# Autodesk Inventor assembly: Leg_joint_roll_pitch
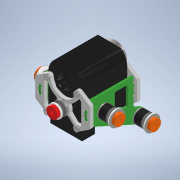
[picture p0: Inventor's stored thumbnail of the model, 180x180]
Saved by Autodesk Inventor 2020 (Build 240168000, 168)
## iProperties
Part Number: Leg_joint_roll_pitch
Document SubType Name: Assembly
Designer: Masato Kubotera
Mass: 101.309 g
Surface Area: 368.925 cm^2
Volume: 74.117 cm^3
Density: 1.36688 g/cm^3
Author: Masato Kubotera
## Documents named in this file (20)
- C:\Users\MasatoKubotera\Documents\Inventor\SUSTAINA-OP\LowerBody\Leg_joint\Leg_joint_roll_pitch.iam
- C:\Users\MasatoKubotera\Documents\Inventor\SUSTAINA-OP\LowerBody\Leg_joint\Leg_joint_pitch_frame.ipt
- C:\Users\MasatoKubotera\Documents\Inventor\SUSTAINA-OP\LowerBody\Leg_joint\Leg_joint_roll_frame.ipt
- C:\Users\MasatoKubotera\Documents\Inventor\SUSTAINA-OP\ReadyMade\Screw\M2_6-20.ipt
- C:\Users\MasatoKubotera\Documents\Inventor\SUSTAINA-OP\ReadyMade\Screw\M2_6-15.ipt
- C:\Users\MasatoKubotera\Documents\Inventor\SUSTAINA-OP\ReadyMade\Bush\80F-0603.ipt
- C:\Users\MasatoKubotera\Documents\Inventor\SUSTAINA-OP\ReadyMade\Washer\CC-0612-50B.ipt
- C:\Users\MasatoKubotera\Documents\Inventor\SUSTAINA-OP\ReadyMade\InsertNut\SF419.ipt
- C:\Users\MasatoKubotera\Documents\Inventor\SUSTAINA-OP\ReadyMade\Washer\UUW-0412-10H.ipt
- C:\Users\MasatoKubotera\Documents\Inventor\SUSTAINA-OP\ReadyMade\Spacer\SLSBF6-39.5-M4-N4.ipt
- C:\Users\MasatoKubotera\Documents\Inventor\SUSTAINA-OP\ReadyMade\Screw\DBTS4-11-6-DHC.ipt
- C:\Users\MasatoKubotera\Documents\Inventor\SUSTAINA-OP\ReadyMade\Screw\DBTS4-5-5-DHC.ipt
- C:\Users\MasatoKubotera\Documents\Inventor\SUSTAINA-OP\ReadyMade\Screw\DBTS4-10-4-DHC.ipt
- C:\Users\MasatoKubotera\Documents\Inventor\SUSTAINA-OP\ReadyMade\InsertNut\S4-05-3W.ipt
- C:\Users\MasatoKubotera\Documents\Inventor\SUSTAINA-OP\ReadyMade\Screw\DBTS4-11-8-DHC.ipt
- C:\Users\MasatoKubotera\Documents\Inventor\SUSTAINA-OP\ReadyMade\Washer\TT-0612-10.ipt
- C:\Users\MasatoKubotera\Documents\Inventor\SUSTAINA-OP\ReadyMade\Washer\TT-0814-10.ipt
- C:\Users\MasatoKubotera\Documents\Inventor\SUSTAINA-OP\ReadyMade\Washer\CCC-0612-65B.ipt
- C:\Users\MasatoKubotera\Documents\Inventor\SUSTAINA-OP\ReadyMade\KONDO\B3M-SC-1170-A_with_ClampHorn.iam
- C:\Users\MasatoKubotera\Documents\Inventor\SUSTAINA-OP\ReadyMade\Washer\UUW-0614-03H.ipt
## Components (50 placed, 19 different names)
1. B3M-SC-1170-A_with_ClampHorn:1 [sub-assembly] — 挿入:246, 挿入:247, 挿入:248, 挿入:249, メイト:18, フラッシュ:10, メイト:19
2. Leg_joint_roll_frame:1 — 挿入:5, 挿入:6, 挿入:7, 挿入:8, 挿入:9, 挿入:10, 角度:1, フラッシュ:2, メイト:3, メイト:4, メイト:5, 挿入:248, 挿入:249
3. Leg_joint_roll_frame:2 — 挿入:15, 挿入:16, 挿入:17, 挿入:18, 角度:2, 角度:4, 挿入:246, 挿入:247
4. Leg_joint_pitch_frame:1 — フラッシュ:3, 挿入:19, フラッシュ:4, メイト:5, 挿入:20, 挿入:21, 挿入:22
5. Leg_joint_pitch_frame:2 — フラッシュ:2, フラッシュ:3, フラッシュ:4, メイト:3, メイト:4, 挿入:23, 挿入:24, 挿入:25, 挿入:26
6. UUW-0412-10H:1 — 挿入:9, 挿入:27
7. UUW-0412-10H:2 — 挿入:17, 挿入:28, 挿入:33
8. UUW-0412-10H:3 — 挿入:19, 挿入:226, 挿入:241
9. UUW-0412-10H:4 — 挿入:22, 挿入:35, 挿入:240
10. UUW-0412-10H:5 — 挿入:23, 挿入:227, 挿入:239
11. UUW-0412-10H:6 — 挿入:26, 挿入:37, 挿入:238
12. UUW-0412-10H:7 — 挿入:27, 挿入:38, 挿入:43
13. SF419:1 — 挿入:25
14. SF419:2 — 挿入:20
15. S4-05-3W:1 — 挿入:10, 角度:1
16. S4-05-3W:2 — 挿入:18, 角度:2
17. SLSBF6-39.5-M4-N4:1 — 挿入:21, 挿入:24, 角度:4
18. DBS4-5-5:1 — 挿入:38, 挿入:232
19. DBTS4-11-6:3 — 挿入:37, 挿入:257
20. DBTS4-11-6:4 — 挿入:35, 挿入:254
21. DBTS4-10-4:1 — 挿入:33, 挿入:233
22. DBTS4-11-8:1 — 挿入:226, 挿入:255
23. DBTS4-11-8:2 — 挿入:227, 挿入:256
24. TT-0612-10:1 — 挿入:233
25. TT-0612-10:2 — 挿入:232
26. TT-0814-10:1 — 挿入:250
27. TT-0814-10:2 — 挿入:251
28. TT-0814-10:3 — 挿入:253
29. TT-0814-10:4 — 挿入:252
30. CCC-0612-65B:1 — 挿入:238, 挿入:245
31. CCC-0612-65B:2 — 挿入:241, 挿入:243
32. CCC-0612-65B:3 — 挿入:239, 挿入:244
33. CCC-0612-65B:4 — 挿入:240, 挿入:242
34. CC-0612-50B:5 — 挿入:28, 挿入:44
35. 80F-0603:1 — 挿入:43
36. 80F-0603:2 — 挿入:44
37. 80F-0603:3 — 挿入:243
38. 80F-0603:4 — 挿入:242
39. 80F-0603:5 — 挿入:244
40. 80F-0603:6 — 挿入:245
41. UUW-0614-03H:1 — 挿入:250, 挿入:256
42. UUW-0614-03H:2 — 挿入:251, 挿入:257
43. UUW-0614-03H:3 — 挿入:253, 挿入:255
44. UUW-0614-03H:4 — 挿入:252, 挿入:254
45. M2_6-20:1 — 挿入:7
46. M2_6-20:2 — 挿入:8
47. M2_6-20:3 — 挿入:5
48. M2_6-20:4 — 挿入:6
49. M2_6-15:2 — 挿入:16
50. M2_6-15:3 — 挿入:15
## Relationships (62: Insert 50, Mate 5, Flush 4, Angle 3)
- 挿入:5 [Insert]: Leg_joint_roll_frame:1 ↔ M2_6-20:3
- 挿入:6 [Insert]: Leg_joint_roll_frame:1 ↔ M2_6-20:4
- 挿入:7 [Insert]: Leg_joint_roll_frame:1 ↔ M2_6-20:1
- 挿入:8 [Insert]: Leg_joint_roll_frame:1 ↔ M2_6-20:2
- 挿入:9 [Insert]: Leg_joint_roll_frame:1 ↔ UUW-0412-10H:1
- 挿入:10 [Insert]: Leg_joint_roll_frame:1 ↔ S4-05-3W:1
- 角度:1 [Angle] (0 deg): Leg_joint_roll_frame:1 ↔ S4-05-3W:1
- 挿入:15 [Insert]: Leg_joint_roll_frame:2 ↔ M2_6-15:3
- 挿入:16 [Insert]: Leg_joint_roll_frame:2 ↔ M2_6-15:2
- 挿入:17 [Insert]: Leg_joint_roll_frame:2 ↔ UUW-0412-10H:2
- 挿入:18 [Insert]: Leg_joint_roll_frame:2 ↔ S4-05-3W:2
- 角度:2 [Angle] (0 deg): Leg_joint_roll_frame:2 ↔ S4-05-3W:2
- 挿入:19 [Insert]: Leg_joint_pitch_frame:1 ↔ UUW-0412-10H:3
- 挿入:20 [Insert]: Leg_joint_pitch_frame:1 ↔ SF419:2
- 挿入:21 [Insert]: Leg_joint_pitch_frame:1 ↔ SLSBF6-39.5-M4-N4:1
- 挿入:22 [Insert]: Leg_joint_pitch_frame:1 ↔ UUW-0412-10H:4
- 挿入:23 [Insert]: Leg_joint_pitch_frame:2 ↔ UUW-0412-10H:5
- 挿入:24 [Insert]: Leg_joint_pitch_frame:2 ↔ SLSBF6-39.5-M4-N4:1
- 挿入:25 [Insert]: Leg_joint_pitch_frame:2 ↔ SF419:1
- 挿入:26 [Insert]: Leg_joint_pitch_frame:2 ↔ UUW-0412-10H:6
- 挿入:27 [Insert]: UUW-0412-10H:1 ↔ UUW-0412-10H:7
- 挿入:28 [Insert]: UUW-0412-10H:2 ↔ CC-0612-50B:5
- 挿入:33 [Insert]: UUW-0412-10H:2 ↔ DBTS4-10-4:1
- 挿入:35 [Insert]: UUW-0412-10H:4 ↔ DBTS4-11-6:4
- 挿入:37 [Insert]: UUW-0412-10H:6 ↔ DBTS4-11-6:3
- 挿入:38 [Insert]: UUW-0412-10H:7 ↔ DBS4-5-5:1
- 挿入:43 [Insert]: UUW-0412-10H:7 ↔ 80F-0603:1
- 挿入:44 [Insert]: CC-0612-50B:5 ↔ 80F-0603:2
- フラッシュ:2 [Flush]: Leg_joint_roll_frame:1 ↔ Leg_joint_pitch_frame:2
- フラッシュ:3 [Flush]: Leg_joint_pitch_frame:1 ↔ Leg_joint_pitch_frame:2
- フラッシュ:4 [Flush]: Leg_joint_pitch_frame:1 ↔ Leg_joint_pitch_frame:2
- メイト:3 [Mate] (0.025 mm): Leg_joint_roll_frame:1 ↔ Leg_joint_pitch_frame:2
- メイト:4 [Mate] (0.025 mm): Leg_joint_roll_frame:1 ↔ Leg_joint_pitch_frame:2
- メイト:5 [Mate] (0.025 mm): Leg_joint_roll_frame:1 ↔ Leg_joint_pitch_frame:1
- 角度:4 [Angle] (0 deg): Leg_joint_roll_frame:2 ↔ SLSBF6-39.5-M4-N4:1
- 挿入:226 [Insert]: UUW-0412-10H:3 ↔ DBTS4-11-8:1
- 挿入:227 [Insert]: UUW-0412-10H:5 ↔ DBTS4-11-8:2
- 挿入:232 [Insert]: DBS4-5-5:1 ↔ TT-0612-10:2
- 挿入:233 [Insert]: DBTS4-10-4:1 ↔ TT-0612-10:1
- 挿入:238 [Insert]: UUW-0412-10H:6 ↔ CCC-0612-65B:1
- 挿入:239 [Insert]: UUW-0412-10H:5 ↔ CCC-0612-65B:3
- 挿入:240 [Insert]: UUW-0412-10H:4 ↔ CCC-0612-65B:4
- 挿入:241 [Insert]: UUW-0412-10H:3 ↔ CCC-0612-65B:2
- 挿入:242 [Insert]: CCC-0612-65B:4 ↔ 80F-0603:4
- 挿入:243 [Insert]: CCC-0612-65B:2 ↔ 80F-0603:3
- 挿入:244 [Insert]: CCC-0612-65B:3 ↔ 80F-0603:5
- 挿入:245 [Insert]: CCC-0612-65B:1 ↔ 80F-0603:6
- 挿入:246 [Insert]: B3M-SC-1170-A_with_ClampHorn:1 ↔ Leg_joint_roll_frame:2
- 挿入:247 [Insert]: B3M-SC-1170-A_with_ClampHorn:1 ↔ Leg_joint_roll_frame:2
- 挿入:248 [Insert]: B3M-SC-1170-A_with_ClampHorn:1 ↔ Leg_joint_roll_frame:1
- 挿入:249 [Insert]: B3M-SC-1170-A_with_ClampHorn:1 ↔ Leg_joint_roll_frame:1
- 挿入:250 [Insert]: TT-0814-10:1 ↔ UUW-0614-03H:1
- メイト:18 [Mate]: B3M-SC-1170-A_with_ClampHorn:1
- フラッシュ:10 [Flush]: B3M-SC-1170-A_with_ClampHorn:1
- メイト:19 [Mate]: B3M-SC-1170-A_with_ClampHorn:1
- 挿入:251 [Insert]: TT-0814-10:2 ↔ UUW-0614-03H:2
- 挿入:252 [Insert]: TT-0814-10:4 ↔ UUW-0614-03H:4
- 挿入:253 [Insert]: TT-0814-10:3 ↔ UUW-0614-03H:3
- 挿入:254 [Insert]: DBTS4-11-6:4 ↔ UUW-0614-03H:4
- 挿入:255 [Insert]: DBTS4-11-8:1 ↔ UUW-0614-03H:3
- 挿入:256 [Insert]: DBTS4-11-8:2 ↔ UUW-0614-03H:1
- 挿入:257 [Insert]: DBTS4-11-6:3 ↔ UUW-0614-03H:2
